# Autodesk Inventor assembly: element_R
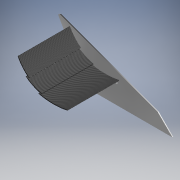
[picture p0: Inventor's stored thumbnail of the model, 180x180]
Saved by Autodesk Inventor 2018.1 (Build 221171000, 171)
## iProperties
Created: 2017-10-22
Part Number: element_R
Material: 一般
Document SubType Name: Assembly
Designer: ku_sk
Author: ku_sk
## Documents named in this file (4)
- D:\kuwano\Documents\Inventor\KITformula\KS-15_Aero_CAD\type4\F-wing\parts\element_side\element_R.iam
- D:\kuwano\Documents\Inventor\KITformula\KS-15_Aero_CAD\type4\F-wing\parts\element_side\parts\element_1.ipt
- D:\kuwano\Documents\Inventor\KITformula\KS-15_Aero_CAD\type4\F-wing\parts\element_side\parts\element_2.ipt
- D:\kuwano\Documents\Inventor\KITformula\KS-15_Aero_CAD\type4\F-wing\parts\element_side\parts\stay_middle.ipt
## Components (4 placed, 3 different names)
1. stay_middle:1 — フラッシュ:17, フラッシュ:18, フラッシュ:19
2. element_1:1
3. element_2:1
4. element_2:2
## Relationships (3: Flush 3)
- フラッシュ:17 [Flush]: stay_middle:1
- フラッシュ:18 [Flush]: stay_middle:1
- フラッシュ:19 [Flush]: stay_middle:1
